# Autodesk Inventor assembly: B-1100-1_MIR
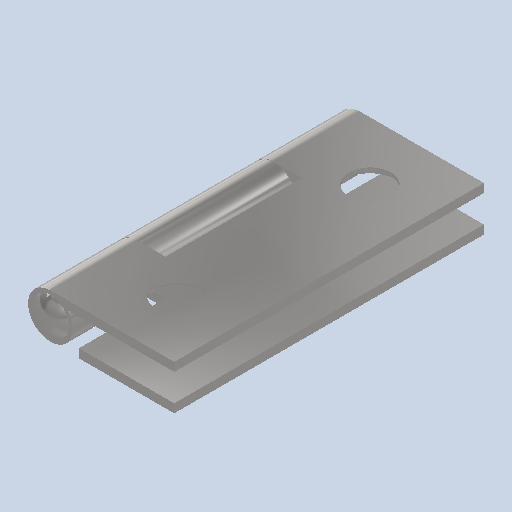
[picture p0: Inventor's stored thumbnail of the model, 512x512]
Saved by Autodesk Inventor 2024 (Build 280153000, 153)
## iProperties
Created: 2008-11-26
Part Number: B-1100-1_MIR
Description: STEP AP203
Document SubType Name: Assembly
Designer: tanoue_kota
Mass: 4.05928 g
Surface Area: 15.1281 cm^2
Volume: 0.50741 cm^3
Density: 8 g/cm^3
Title: B-1100-1.STEP
Revision Number: ANY
Sending System: SolidWorks 2007
Preprocessor: SwSTEP 2.0
## Documents named in this file (4)
- C:\Users\田之上巧太\Documents\Inventor\キャチロボ2023\BasicParts\Hinge\B-1100-1\B-1100-1_MIR.iam
- C:\Users\田之上巧太\Documents\Inventor\キャチロボ2023\BasicParts\Hinge\B-1100-1\B-1100-1qWB__ÃÞÌ«ÙÄ_MIR.ipt
- C:\Users\田之上巧太\Documents\Inventor\キャチロボ2023\BasicParts\Hinge\B-1100-1\B-1100-1qWA__ÃÞÌ«ÙÄ_MIR.ipt
- C:\Users\田之上巧太\Documents\Inventor\キャチロボ2023\BasicParts\Hinge\B-1100-1\B-1100-1Vtg__ÃÞÌ«ÙÄ_MIR.ipt
## Components (3 placed, 3 different names)
1. B-1100-1qWB__ÃÞÌ«ÙÄ_MIR:1 — フラッシュ:2, フラッシュ:1, メイト:1, 回転:1
2. B-1100-1qWA__ÃÞÌ«ÙÄ_MIR:1 — フラッシュ:2, フラッシュ:1, メイト:1, 回転:1, 回転:2
3. B-1100-1Vtg__ÃÞÌ«ÙÄ_MIR:1 — 回転:2
## Relationships (5: Flush 2, RevoluteJoint 2, Mate 1)
- フラッシュ:2 [Flush]: B-1100-1qWB__ÃÞÌ«ÙÄ_MIR:1 ↔ B-1100-1qWA__ÃÞÌ«ÙÄ_MIR:1
- フラッシュ:1 [Flush]: B-1100-1qWB__ÃÞÌ«ÙÄ_MIR:1 ↔ B-1100-1qWA__ÃÞÌ«ÙÄ_MIR:1
- メイト:1 [Mate]: B-1100-1qWB__ÃÞÌ«ÙÄ_MIR:1 ↔ B-1100-1qWA__ÃÞÌ«ÙÄ_MIR:1
- 回転:1 [RevoluteJoint]: B-1100-1qWB__ÃÞÌ«ÙÄ_MIR:1 ↔ B-1100-1qWA__ÃÞÌ«ÙÄ_MIR:1
- 回転:2 [RevoluteJoint]: B-1100-1qWA__ÃÞÌ«ÙÄ_MIR:1 ↔ B-1100-1Vtg__ÃÞÌ«ÙÄ_MIR:1
